# Autodesk Inventor assembly: AKM2G-51X-ACDNCA00
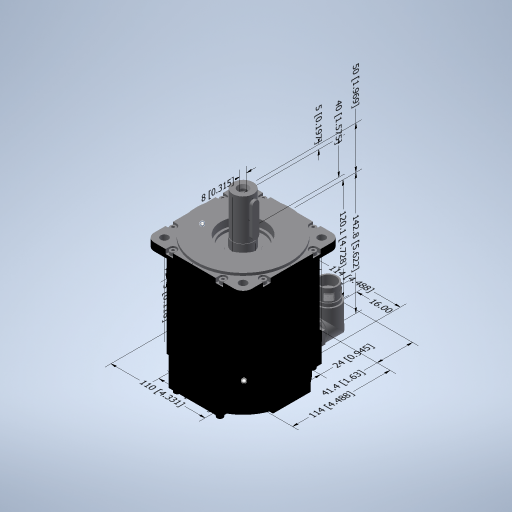
[picture p0: Inventor's stored thumbnail of the model, 512x512]
Saved by Autodesk Inventor 2024 (Build 280153000, 153)
## iProperties
Created: 2024-01-26
Part Number: AKM2G-51X-ACDNCA00
Catalog Web Link: www.cadenas.de
Description: AKM2G Size 5-AKM2G Series
Vendor: KOLLMORGEN
Document SubType Name: Assembly
Designer: psAdmin
Manufacturer: KOLLMORGEN
Mass: 1626.42 g
Surface Area: 1508.58 cm^2
Volume: 1626.42 cm^3
Density: 1 g/cm^3
Category: PARTsolutions
Company: KOLLMORGEN
PSOL_IDENT_0: {$CADENAS_DATA/23d-libs/kollmorgen/akm2g/parts/akm2g5_asmtab.prj},220 {VTYP=3D},{STYP=ASSTAB},{NB=AK
PSOL_IDENT_1: M2G-51X-ACDNCA00},{LINA=AKM2G-51X-ACDNCA00},{NN=AKM2G Size 5},{DATE=23.06.2022 07:51:32},{GEOMDATE=0
PSOL_IDENT_2: 2.03.2021 06:09:44},{VERSION=},{LINEID=10},{WBVAR=SL,MO,SH,CON,BR,FD,TS,SS},{WBNUMERIC=}  {NB=AKM2G-
PSOL_IDENT_3: 51X-ACDNCA00},{LINA=AKM2G-51X-ACDNCA00},{KT=DUMMY},{PN=AKM2G-51X-ACDNCA00},{FS=5 = Size 5},{SL=1},{W=
PSOL_IDENT_4: X},{MO=A},{SH=C},{CON=D},{BR=N},{FD=CA},{TS=0},{SS=0},{FDALG=  'CA' , 'CA = SFD3 Smart Feedback', 'G
PSOL_IDENT_5: U' , 'GU = MT Hiperface DSL'  , 'LD', 'LD = MT Inductive Endat 2.2'  },{RL=30.3},{PPATH=akm2g5_asmtp
PSOL_IDENT_6: l.prj},{FDPN=CA},{TSALG= '0', '0 = Standard (pt-1000 + Avalanche ptc in Series)' },{FDH=0},{C=9},{D=
PSOL_IDENT_7: 110},{E=130},{H=M8},{J=24},{K=50},{L=142.8},{P=27},{R=8},{S=5},{T=40},{X=120.1}
NB: AKM2G-51X-ACDNCA00
NN: AKM2G Size 5
NT: AKM2G Series
NBSYN: $PN.
LINA: AKM2G-51X-ACDNCA00
CATALOG: Kollmorgen
PN: AKM2G-51X-ACDNCA00
FS: 5 = Size 5
SL: 1 = 1 Stack
W: X
MO: A = Metric IEC
SH: C = Closed Keyway
CON: D = Single Right Angle M23
BR: N = No Brake
FD: CA = SFD3 Smart Feedback
TS: 0 = Standard (pt-1000 + Avalanche ptc in Series)
SS: 0 = No seal
C: 9
D: 110
E: 130
H: M8
J: 24
K: 50
L: 142.8
P: 27
R: 8
S: 5
T: 40
X: 120.1
SUPPLIER: KOLLMORGEN
ARTICLENO: AKM2G-51X-ACDNCA00
BOMINFO: AKM2G-51X-ACDNCA00
CREATOR: CADENAS GmbH
Title: AKM2G-51X-ACDNCA00
Author: Cadenas PARTsolutions
Comments: AKM2G Series
## Documents named in this file (5)
- C:\Users\Owner\PycharmProjects\DodgeBot\CAD_FILES\AKM2G-51X-ACDNCA00.iam
- C:\Users\Owner\PycharmProjects\DodgeBot\CAD_FILES\AKM2G-51DNCA_R.ipt
- C:\Users\Owner\PycharmProjects\DodgeBot\CAD_FILES\AKM2G-51DNCA_H.ipt
- C:\Users\Owner\PycharmProjects\DodgeBot\CAD_FILES\AKM2G-5ACDNCA_F.ipt
- C:\Users\Owner\PycharmProjects\DodgeBot\CAD_FILES\Connector-41,4D-c.ipt
## Components (4 placed, 4 different names)
1. AKM2G-51DNCA_R:1 — R_XY@1 <-> H1_XY@2, R_Z@1 <-> H1_Z@2, R_YZ@1 <-> H1_YZ@2, CON2_XY@1 <-> to_XY@4, CON2_Z@1 <-> to_Z@4, CON2_YZ@1 <-> to_YZ@4
2. AKM2G-51DNCA_H:1 — R_XY@1 <-> H1_XY@2, R_Z@1 <-> H1_Z@2, R_YZ@1 <-> H1_YZ@2, H2_XY@2 <-> F_XY@3, H2_Z@2 <-> F_Z@3, H2_YZ@2 <-> F_YZ@3
3. AKM2G-5ACDNCA_F:1 — H2_XY@2 <-> F_XY@3, H2_Z@2 <-> F_Z@3, H2_YZ@2 <-> F_YZ@3
4. Connector-41,4D-c:1 — CON2_XY@1 <-> to_XY@4, CON2_Z@1 <-> to_Z@4, CON2_YZ@1 <-> to_YZ@4
## Relationships (9: Mate 6, Angle 3)
- R_XY@1 <-> H1_XY@2 [Mate]: AKM2G-51DNCA_R:1 ↔ AKM2G-51DNCA_H:1
- R_Z@1 <-> H1_Z@2 [Mate]: AKM2G-51DNCA_R:1 ↔ AKM2G-51DNCA_H:1
- R_YZ@1 <-> H1_YZ@2 [Angle] (0 deg): AKM2G-51DNCA_R:1 ↔ AKM2G-51DNCA_H:1
- H2_XY@2 <-> F_XY@3 [Mate]: AKM2G-51DNCA_H:1 ↔ AKM2G-5ACDNCA_F:1
- H2_Z@2 <-> F_Z@3 [Mate]: AKM2G-51DNCA_H:1 ↔ AKM2G-5ACDNCA_F:1
- H2_YZ@2 <-> F_YZ@3 [Angle] (0 deg): AKM2G-51DNCA_H:1 ↔ AKM2G-5ACDNCA_F:1
- CON2_XY@1 <-> to_XY@4 [Mate]: AKM2G-51DNCA_R:1 ↔ Connector-41,4D-c:1
- CON2_Z@1 <-> to_Z@4 [Mate]: AKM2G-51DNCA_R:1 ↔ Connector-41,4D-c:1
- CON2_YZ@1 <-> to_YZ@4 [Angle] (90 deg): AKM2G-51DNCA_R:1 ↔ Connector-41,4D-c:1
